# Autodesk Inventor assembly: dribler
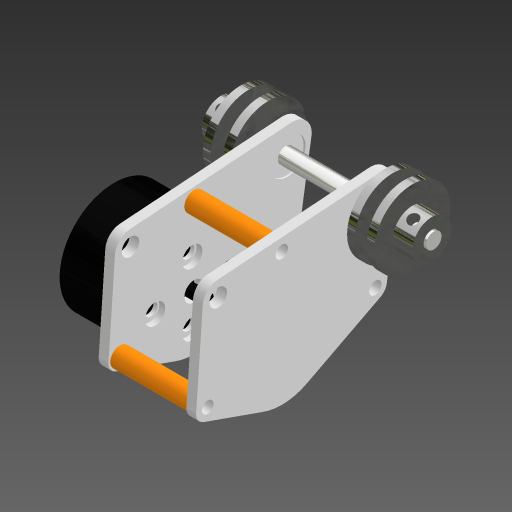
[picture p0: Inventor's stored thumbnail of the model, 512x512]
Saved by Autodesk Inventor 2023 (Build 270158000, 158)
## iProperties
Created: 2025-07-07
Part Number: dribler
Document SubType Name: Assembly
Designer: daa
Author: daa
## Documents named in this file (8)
- C:\Users\daa\Documents\DASH_V2\dribler.iam
- C:\Users\daa\Documents\DASH_V2\Dribler_v2\drib_lef.ipt
- C:\Users\daa\Documents\DASH_V2\Dribler_v2\drib_rig.ipt
- C:\Users\daa\Documents\DASH_V2\Dribler_v2\motor_c2822.ipt
- C:\Users\daa\Documents\DASH_V2\Dribler_v2\rack.ipt
- C:\Users\daa\Documents\DASH_V2\Dribler_v2\koleso_left.ipt
- C:\Users\daa\Documents\DASH_V2\Dribler_v2\bearing.ipt
- C:\Users\daa\Documents\DASH_V2\Dribler_v2\axis.ipt
## Components (11 placed, 7 different names)
1. drib_lef:1 — С поворотом:2, С поворотом:7
2. drib_rig:1 — С поворотом:1, С поворотом:3, С поворотом:4, С поворотом:5, С поворотом:6
3. motor_c2822:1 — С поворотом:1
4. rack:1 — С поворотом:6
5. koleso_left:1 — С поворотом:8
6. koleso_left:2 — С поворотом:9
7. bearing:1 — С поворотом:3, С поворотом:8
8. bearing:2 — С поворотом:2, С поворотом:9, Жесткий:1
9. rack:2 — С поворотом:4, С поворотом:7
10. rack:3 — С поворотом:5
11. axis:1 — Жесткий:1
## Relationships (10: RevoluteJoint 9, WeldJoint 1)
- С поворотом:1 [RevoluteJoint]: drib_rig:1 ↔ motor_c2822:1
- С поворотом:2 [RevoluteJoint] (2 mm): drib_lef:1 ↔ bearing:2
- С поворотом:3 [RevoluteJoint] (-2 mm): drib_rig:1 ↔ bearing:1
- С поворотом:4 [RevoluteJoint]: drib_rig:1 ↔ rack:2
- С поворотом:5 [RevoluteJoint]: drib_rig:1 ↔ rack:3
- С поворотом:6 [RevoluteJoint]: drib_rig:1 ↔ rack:1
- С поворотом:7 [RevoluteJoint]: drib_lef:1 ↔ rack:2
- С поворотом:8 [RevoluteJoint]: koleso_left:1 ↔ bearing:1
- С поворотом:9 [RevoluteJoint]: koleso_left:2 ↔ bearing:2
- Жесткий:1 [WeldJoint] (-17 mm): bearing:2 ↔ axis:1
